# Autodesk Inventor assembly: 皿
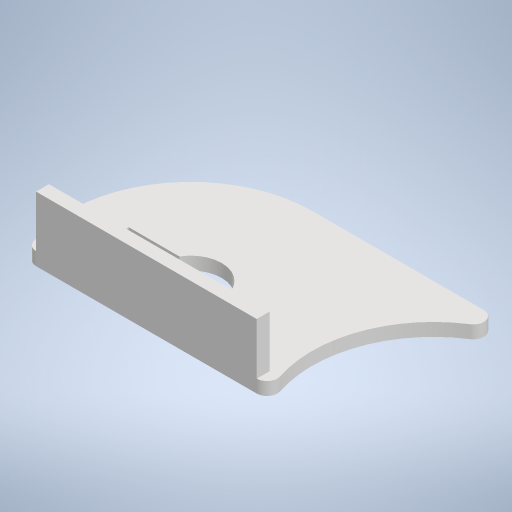
[picture p0: Inventor's stored thumbnail of the model, 512x512]
Saved by Autodesk Inventor 2024.1 (Build 281209000, 209)
## iProperties
Created: 2024-05-01
Part Number: 皿
Document SubType Name: Assembly
Designer: hibik
Author: hibik
## Documents named in this file (3)
- C:\Users\hibik\Desktop\ロボメカ\2年\新歓\ベルトコンベア\皿.iam
- C:\Users\hibik\Desktop\ロボメカ\2年\新歓\ベルトコンベア\皿.ipt
- C:\Users\hibik\Desktop\ロボメカ\2年\新歓\ベルトコンベア\皿_壁.ipt
## Components (2 placed, 2 different names)
1. 皿:1 — メイト:1, フラッシュ:1, メイト:2
2. 皿_壁:1 — メイト:1, フラッシュ:1, メイト:2
## Relationships (3: Mate 2, Flush 1)
- メイト:1 [Mate]: 皿:1 ↔ 皿_壁:1
- フラッシュ:1 [Flush]: 皿:1 ↔ 皿_壁:1
- メイト:2 [Mate]: 皿:1 ↔ 皿_壁:1
